# Autodesk Inventor assembly: 2020LongRobotV06
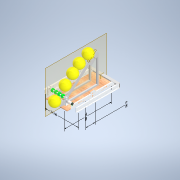
[picture p0: Inventor's stored thumbnail of the model, 180x180]
Saved by Autodesk Inventor 2020.2 (Build 242310000, 310)
## iProperties
Created: 2020-01-25
Part Number: 2020LongRobotV06
Document SubType Name: Assembly
Designer: robst
Author: robst
## Documents named in this file (11)
- C:\git\CAD-Development\robSteele\ShapeWays\KindleStand\2020LongRobotV06.iam
- C:\git\CAD-Development\robSteele\2020LongRobotBase\2020 Wood BaseV04.ipt
- C:\git\CAD-Development\robSteele\2020LongRobotBase\2020 End Plate.ipt
- C:\git\CAD-Development\robSteele\2020LongRobotBase\am-3922 AM14U4 Inside Plate.ipt
- C:\git\CAD-Development\robSteele\2020LongRobotBase\am-3921 AM14U4 Outside Plate.ipt
- C:\git\CAD-Development\robSteele\2020LongRobotBase\ballRampWithPocketForPowerCell.ipt
- C:\git\CAD-Development\robSteele\2020LongRobotBase\am-3922 AM14U4 Inside Plate_MIR.ipt
- C:\git\CAD-Development\robSteele\2020LongRobotBase\am-3921 AM14U4 Outside Plate_MIR.ipt
- C:\git\CAD-Development\robSteele\2020LongRobotBase\ballRampWithPocketForPowerCell_MIR1.ipt
- C:\git\CAD-Development\robSteele\2020LongRobotBase\am-3312a_Gear Intake Kit Gear Config.iam
- C:\git\CAD-Development\robSteele\2020LongRobotBase\1892-YEL.ipt
## Components (14 placed, 10 different names)
1. 2020 Wood BaseV04:1 — Flush:1, Flush:2, Flush:3, Mate:1, Mate:3, Mate:6, Mate:7, Mate:11, Flush:8
2. 2020 End Plate:1 — Flush:4, Mate:1, Mate:2, Mate:5
3. am-3922 AM14U4 Inside Plate:1 — Mate:2, Mate:3, Mate:4, Flush:5
4. am-3921 AM14U4 Outside Plate:1 — Mate:4, Mate:5, Flush:5
5. ballRampWithPocketForPowerCell:1 — Mate:6, Mate:7, Mate:8, Mate:13, Mate:14, Mate:15, Mate:16, Mate:22, Mate:23
6. am-3922 AM14U4 Inside Plate_MIR:1 — Flush:6, Mate:9
7. am-3921 AM14U4 Outside Plate_MIR:1 — Flush:6, Mate:9
8. ballRampWithPocketForPowerCell_MIR1:1 — Flush:7
9. am-3312a_Gear Intake Kit Gear Config:1 [sub-assembly] — Mate:10, Mate:11, Flush:8
10. 1892-YEL:1 — Mate:12, Mate:13, Mate:17
11. 1892-YEL:2 — Mate:14, Mate:18
12. 1892-YEL:3 — Mate:15, Mate:19
13. 1892-YEL:4 — Mate:16, Mate:20
14. 1892-YEL:5 — Mate:21, Mate:22, Mate:23
## Relationships (31: Mate 23, Flush 8)
- Flush:1: 2020 Wood BaseV04:1
- Flush:2: 2020 Wood BaseV04:1
- Flush:3: 2020 Wood BaseV04:1
- Flush:4: 2020 End Plate:1
- Mate:1: 2020 Wood BaseV04:1 ↔ 2020 End Plate:1
- Mate:2: 2020 End Plate:1 ↔ am-3922 AM14U4 Inside Plate:1
- Mate:3: 2020 Wood BaseV04:1 ↔ am-3922 AM14U4 Inside Plate:1
- Mate:4 (85.725 mm): am-3922 AM14U4 Inside Plate:1 ↔ am-3921 AM14U4 Outside Plate:1
- Mate:5: 2020 End Plate:1 ↔ am-3921 AM14U4 Outside Plate:1
- Flush:5: am-3922 AM14U4 Inside Plate:1 ↔ am-3921 AM14U4 Outside Plate:1
- Mate:6: 2020 Wood BaseV04:1 ↔ ballRampWithPocketForPowerCell:1
- Mate:7: 2020 Wood BaseV04:1 ↔ ballRampWithPocketForPowerCell:1
- Mate:8 (57.15 mm): ballRampWithPocketForPowerCell:1
- Flush:6: am-3922 AM14U4 Inside Plate_MIR:1 ↔ am-3921 AM14U4 Outside Plate_MIR:1
- Mate:9 (85.725 mm): am-3922 AM14U4 Inside Plate_MIR:1 ↔ am-3921 AM14U4 Outside Plate_MIR:1
- Flush:7 (-57.15 mm): ballRampWithPocketForPowerCell_MIR1:1
- Mate:10: am-3312a_Gear Intake Kit Gear Config:1
- Mate:11 (63.5 mm): 2020 Wood BaseV04:1 ↔ am-3312a_Gear Intake Kit Gear Config:1
- Flush:8: 2020 Wood BaseV04:1 ↔ am-3312a_Gear Intake Kit Gear Config:1
- Mate:12: 1892-YEL:1
- Mate:13: ballRampWithPocketForPowerCell:1 ↔ 1892-YEL:1
- Mate:14: ballRampWithPocketForPowerCell:1 ↔ 1892-YEL:2
- Mate:15: ballRampWithPocketForPowerCell:1 ↔ 1892-YEL:3
- Mate:16: ballRampWithPocketForPowerCell:1 ↔ 1892-YEL:4
- Mate:17: 1892-YEL:1
- Mate:18: 1892-YEL:2
- Mate:19: 1892-YEL:3
- Mate:20: 1892-YEL:4
- Mate:21: 1892-YEL:5
- Mate:22: ballRampWithPocketForPowerCell:1 ↔ 1892-YEL:5
- Mate:23: ballRampWithPocketForPowerCell:1 ↔ 1892-YEL:5
